# Autodesk Inventor assembly: !Structure
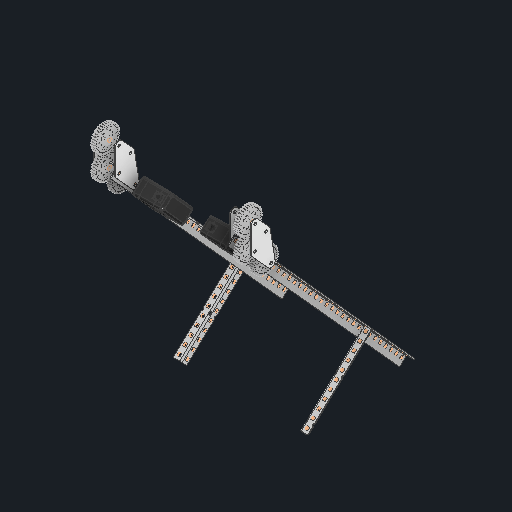
[picture p0: Inventor's stored thumbnail of the model, 512x512]
Saved by Autodesk Inventor 2025 (Build 290162000, 162)
## iProperties
Created: 2024-12-30
Part Number: !Structure
Document SubType Name: Assembly
Designer: Averey Ku
Author: Averey Ku
## Documents named in this file (7)
- D:\VEX\High Stakes\CAD\V4\Lady Brown\Structure\!Structure.iam
- D:\VEX\High Stakes\CAD\ROBOPROS-CAD-Inventor\Structure\C Channel\Aluminum 1x3x1 Half Thick Cut\Alu C Half Thick 1x3x1x32.ipt
- D:\VEX\High Stakes\CAD\ROBOPROS-CAD-Inventor\Structure\Angle\Aluminum 1x1\Alu Angle 1x1x12.ipt
- D:\VEX\High Stakes\CAD\ROBOPROS-CAD-Inventor\Structure\Angle\Aluminum 1x1\Alu Angle 1x1x11.ipt
- D:\VEX\High Stakes\CAD\V4\Lady Brown\Structure\Custom Parts\Gearbox.ipt
- D:\VEX\High Stakes\CAD\ROBOPROS-CAD-Inventor\Modified Parts\Equal Half Cut HS 36T Gear, No Insert.ipt
- D:\VEX\High Stakes\CAD\ROBOPROS-CAD-Inventor\Electronics\V5 Motor (5.5W).ipt
## Components (18 placed, 6 different names)
1. Alu C Half Thick 1x3x1x32:1 — Insert:2, Insert:3, Insert:4, Mate:3, Insert:5, Insert:6, Mate:4, Flush:1
2. Alu Angle 1x1x12:1 — Mate:2
3. Alu Angle 1x1x11:1 — Insert:2, Mate:2
4. Gearbox:1 — Insert:3, Mate:3, Insert:7, Mate:5
5. Equal Half Cut HS 36T Gear, No Insert:1 — Insert:5, Insert:8
6. Equal Half Cut HS 36T Gear, No Insert:2 — Insert:4
7. V5 Motor (5.5W):1 — Insert:6, Mate:4
8. Equal Half Cut HS 36T Gear, No Insert:3 — Insert:7
9. Gearbox:2 — Insert:8, Mate:5
10. Alu C Half Thick 1x3x1x32:2 — Mate:6, Insert:9, Mate:7, Insert:10, Insert:12, Insert:13, Mate:10, Insert:14, Insert:15, Mate:12
11. Alu Angle 1x1x12:2 — Insert:9, Mate:7, Mate:8
12. Alu Angle 1x1x11:2 — Mate:8, Insert:10
13. Equal Half Cut HS 36T Gear, No Insert:4 — Insert:12, Insert:16
14. Equal Half Cut HS 36T Gear, No Insert:5 — Insert:13
15. V5 Motor (5.5W):2 — Mate:10, Insert:14
16. Equal Half Cut HS 36T Gear, No Insert:6
17. Gearbox:3 — Insert:16
18. Gearbox:4 — Insert:15, Mate:12
## Relationships (27: Insert 15, Mate 11, Flush 1)
- [Mate]: Alu C Half Thick 1x3x1x32:1 ↔ Alu Angle 1x1x12:1
- [Insert]: Alu C Half Thick 1x3x1x32:1 ↔ Alu Angle 1x1x12:1
- Insert:2: Alu C Half Thick 1x3x1x32:1 ↔ Alu Angle 1x1x11:1
- Mate:2: Alu Angle 1x1x12:1 ↔ Alu Angle 1x1x11:1
- Insert:3: Alu C Half Thick 1x3x1x32:1 ↔ Gearbox:1
- Insert:4 (12.7 mm): Alu C Half Thick 1x3x1x32:1 ↔ Equal Half Cut HS 36T Gear, No Insert:2
- Mate:3: Alu C Half Thick 1x3x1x32:1 ↔ Gearbox:1
- Insert:5 (12.7 mm): Alu C Half Thick 1x3x1x32:1 ↔ Equal Half Cut HS 36T Gear, No Insert:1
- Insert:6: Alu C Half Thick 1x3x1x32:1 ↔ V5 Motor (5.5W):1
- Mate:4: Alu C Half Thick 1x3x1x32:1 ↔ V5 Motor (5.5W):1
- Insert:7 (14.2875 mm): Gearbox:1 ↔ Equal Half Cut HS 36T Gear, No Insert:3
- Insert:8 (3.7592 mm): Equal Half Cut HS 36T Gear, No Insert:1 ↔ Gearbox:2
- Mate:5: Gearbox:1 ↔ Gearbox:2
- Flush:1 (92.4941 mm): Alu C Half Thick 1x3x1x32:1
- Mate:6 (92.4941 mm): Alu C Half Thick 1x3x1x32:2
- Insert:9: Alu C Half Thick 1x3x1x32:2 ↔ Alu Angle 1x1x12:2
- Mate:7: Alu C Half Thick 1x3x1x32:2 ↔ Alu Angle 1x1x12:2
- Mate:8: Alu Angle 1x1x12:2 ↔ Alu Angle 1x1x11:2
- Insert:10: Alu C Half Thick 1x3x1x32:2 ↔ Alu Angle 1x1x11:2
- Insert:12 (12.7 mm): Alu C Half Thick 1x3x1x32:2 ↔ Equal Half Cut HS 36T Gear, No Insert:4
- Insert:13 (12.7 mm): Alu C Half Thick 1x3x1x32:2 ↔ Equal Half Cut HS 36T Gear, No Insert:5
- Mate:10: Alu C Half Thick 1x3x1x32:2 ↔ V5 Motor (5.5W):2
- Insert:14: Alu C Half Thick 1x3x1x32:2 ↔ V5 Motor (5.5W):2
- [Mate]: Gearbox:3 ↔ Gearbox:4
- Insert:15: Alu C Half Thick 1x3x1x32:2 ↔ Gearbox:4
- Mate:12: Alu C Half Thick 1x3x1x32:2 ↔ Gearbox:4
- Insert:16 (3.7592 mm): Equal Half Cut HS 36T Gear, No Insert:4 ↔ Gearbox:3
## Named parameters: d31_d13 = 0 mm
